# Autodesk Inventor assembly: NEWASS
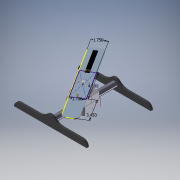
[picture p0: Inventor's stored thumbnail of the model, 180x180]
Saved by Autodesk Inventor 2016 (Build 200138000, 138)
## iProperties
Created: 2017-12-21
Part Number: NEWASS
Document SubType Name: Assembly
Designer: student
Author: student
## Documents named in this file (11)
- C:\Users\student\Documents\GitHub\POV2017\INVENTOR\NEWASS.iam
- C:\Users\student\Documents\GitHub\POV2017\INVENTOR\basemotor.ipt
- C:\Users\student\Documents\GitHub\POV2017\INVENTOR\Rod.ipt
- C:\Users\student\Documents\GitHub\POV2017\INVENTOR\holder.ipt
- C:\Users\student\Documents\GitHub\POV2017\INVENTOR\mOTORHOLDER.ipt
- C:\Users\student\Documents\Inventor\Content Center Files\R2016\en-US\ANSI B18.3.1M(1)\ANSI B18.3.1M - M4x0.7 x 60(2).ipt
- C:\Users\student\Documents\Inventor\Content Center Files\R2016\en-US\AS 1237 (2.1)\AS 1237 - 4.ipt
- C:\Users\student\Documents\Inventor\Content Center Files\R2016\en-US\CNS 4373\CNS 4373 - M 4.ipt
- C:\Users\student\Documents\GitHub\POV2017\INVENTOR\motor.ipt
- C:\Users\student\Documents\GitHub\POV2017\INVENTOR\Assembly1.iam
- C:\Users\student\Documents\GitHub\POV2017\INVENTOR\Lower Power.ipt
## Components (12 placed, 10 different names)
1. basemotor:1 — Rigid:1, Rigid:3, Rigid:5, Rigid:6, Flush:1
2. Rod:1 — Rigid:3, Rigid:4
3. Rod:2 — Rigid:1, Rigid:2
4. holder:1 — Rigid:4
5. holder:2 — Rigid:2
6. mOTORHOLDER:1 — Rigid:5, Rigid:6, Mate:1, Mate:2, Mate:4, Mate:5
7. Broached Socket Head Cap Screw - Metric M4x0.7 x 60:1 — Mate:1, Mate:2, Mate:3
8. AS 1237 (2.1) 4:1 — Mate:3, Mate:4, Insert:1
9. CNS 4373 M 4:1 — Insert:1
10. motor:1 — Mate:5, Flush:1, Rotational:1, Mate:6, Mate:7
11. Assembly1:1 [sub-assembly] — Rotational:1
12. Lower Power:1 — Mate:6, Mate:7
## Relationships (16: Mate 7, WeldJoint 6, Insert 1, Flush 1, RevoluteJoint 1)
- Rigid:1 [WeldJoint]: basemotor:1 ↔ Rod:2
- Rigid:2 [WeldJoint]: Rod:2 ↔ holder:2
- Rigid:3 [WeldJoint]: basemotor:1 ↔ Rod:1
- Rigid:4 [WeldJoint]: Rod:1 ↔ holder:1
- Rigid:5 [WeldJoint]: basemotor:1 ↔ mOTORHOLDER:1
- Rigid:6 [WeldJoint]: basemotor:1 ↔ mOTORHOLDER:1
- Mate:1: mOTORHOLDER:1 ↔ Broached Socket Head Cap Screw - Metric M4x0.7 x 60:1
- Mate:2: mOTORHOLDER:1 ↔ Broached Socket Head Cap Screw - Metric M4x0.7 x 60:1
- Mate:3: Broached Socket Head Cap Screw - Metric M4x0.7 x 60:1 ↔ AS 1237 (2.1) 4:1
- Mate:4: mOTORHOLDER:1 ↔ AS 1237 (2.1) 4:1
- Insert:1: AS 1237 (2.1) 4:1 ↔ CNS 4373 M 4:1
- Mate:5: mOTORHOLDER:1 ↔ motor:1
- Flush:1: basemotor:1 ↔ motor:1
- Rotational:1 [RevoluteJoint]: motor:1 ↔ Assembly1:1
- Mate:6: motor:1 ↔ Lower Power:1
- Mate:7: motor:1 ↔ Lower Power:1
